# Autodesk Inventor assembly: SpringSamsungGalaxySAssy
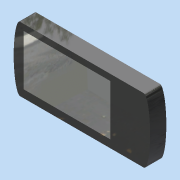
[picture p0: Inventor's stored thumbnail of the model, 180x180]
Saved by Autodesk Inventor 2011 SP1 (Build 150282100, 282)
## iProperties
Created: 2011-08-14
Part Number: SpringSamsungGalaxySAssy
Document SubType Name: Assembly
Designer: dgitz
Author: dgitz
## Documents named in this file (3)
- C:\Dropbox\ICARUS\Remote Control Unit (RCU)\RCU v2\Design\Library\SpringSamsungGalaxySAssy.iam
- C:\Dropbox\ICARUS\Remote Control Unit (RCU)\RCU v2\Design\Library\SprintSamsuingGalaxyS\SprintSamsungGalaxyS.ipt
- C:\Dropbox\ICARUS\Remote Control Unit (RCU)\RCU v2\Design\Library\SprintSamsuingGalaxyS\FacePlate.ipt
## Components (2 placed, 2 different names)
1. SprintSamsungGalaxyS:1 — Mate:1, Mate:2, Mate:3
2. FacePlate:1 — Mate:1, Mate:2, Mate:3
## Relationships (3: Mate 3)
- Mate:1: SprintSamsungGalaxyS:1 ↔ FacePlate:1
- Mate:2: SprintSamsungGalaxyS:1 ↔ FacePlate:1
- Mate:3: SprintSamsungGalaxyS:1 ↔ FacePlate:1
